# Autodesk Inventor assembly: ASY PRS 1200-52 FDS way 2
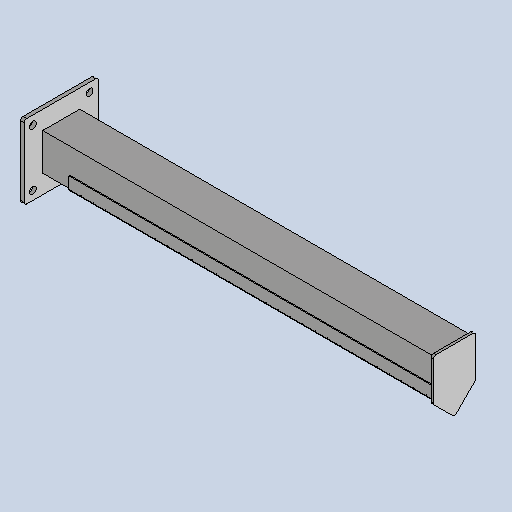
[picture p0: Inventor's stored thumbnail of the model, 512x512]
Saved by Autodesk Inventor 2025.3 (Build 293356030, 356C)
## iProperties
Created: 2025-07-02
Part Number: ASY PRS 1200-52 FDS way 2
Document SubType Name: Assembly
Designer: admin
Author: user
## Documents named in this file (5)
- C:\Users\pokla\Documents\Inventor\PRS-Purovskii\Model\PRS-filter 1200\ASY PRS 1200-52 FDS way 2.iam
- C:\Users\pokla\Documents\Inventor\PRS-Purovskii\Model\PRS-filter 1200\PRS 1200-52-02 FDS 1000 way tube 2.ipt
- C:\Users\pokla\Documents\Inventor\PRS-Purovskii\Model\PRS-filter 1200\PRS 1200-52-03 FDS 1000 CUP 1.ipt
- C:\Users\pokla\Documents\Inventor\PRS-Purovskii\Model\PRS-filter 1200\PRS 1200-52-04 FDS Way FLANGE.ipt
- C:\Users\pokla\Documents\Inventor\PRS-Purovskii\Model\PRS-filter 1200\PRS 1200-52-01 roof 3.ipt
## Components (4 placed, 4 different names)
1. PNS 1662 FDS 1000 way tube 2.ipt:1 — Rigid:10, Rigid:11, Rigid:12
2. PNS 1666 FDS 1000 CUP 1.ipt:1 — Rigid:10
3. SLM 1425 FDS Way FLANGE:1 — Rigid:11
4. NDA-513 roof 3:1 — Rigid:12
## Relationships (3: WeldJoint 3)
- Rigid:10 [WeldJoint]: PNS 1662 FDS 1000 way tube 2.ipt:1 ↔ PNS 1666 FDS 1000 CUP 1.ipt:1
- Rigid:11 [WeldJoint]: PNS 1662 FDS 1000 way tube 2.ipt:1 ↔ SLM 1425 FDS Way FLANGE:1
- Rigid:12 [WeldJoint]: PNS 1662 FDS 1000 way tube 2.ipt:1 ↔ NDA-513 roof 3:1
